# Autodesk Inventor assembly: Manfrotto Logo 01
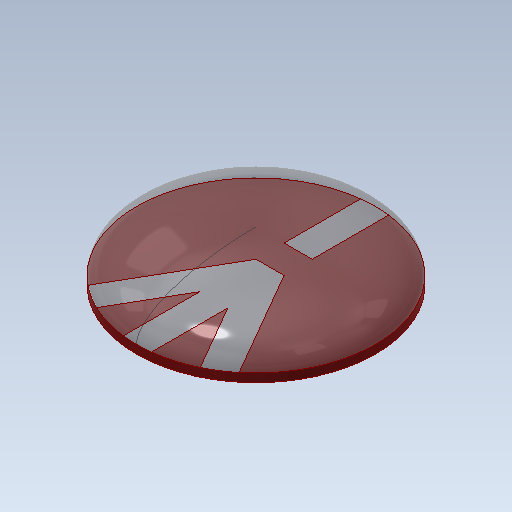
[picture p0: Inventor's stored thumbnail of the model, 512x512]
Saved by Autodesk Inventor 2020 (Build 240168000, 168)
## iProperties
Created: 2012-11-06
Part Number: Manfrotto Logo 01
Document SubType Name: Assembly
Designer: Lance
Mass: 0.140728 g
Surface Area: 2.47849 cm^2
Volume: 0.0737688 cm^3
Density: 1.90769 g/cm^3
Author: Lance
## Documents named in this file (3)
- C:\Users\Hesekiel\Desktop\MUM\Mechanika\Mechanizm elewacji i elektronika Filip\CAD\manfrotto-494rc2-tripod-head.snapshot.1\Manfrotto 494RC2 - Tripod Head\Manfrotto Logo 01.iam
- C:\Users\Hesekiel\Desktop\MUM\Mechanika\Mechanizm elewacji i elektronika Filip\CAD\manfrotto-494rc2-tripod-head.snapshot.1\Manfrotto 494RC2 - Tripod Head\Manfrotto Logo 01 - 1.ipt
- C:\Users\Hesekiel\Desktop\MUM\Mechanika\Mechanizm elewacji i elektronika Filip\CAD\manfrotto-494rc2-tripod-head.snapshot.1\Manfrotto 494RC2 - Tripod Head\Manfrotto Logo 01 - 2.ipt
## Components (2 placed, 2 different names)
1. Manfrotto Logo 01 - 1:1 — Insert:1, Angle:1
2. Manfrotto Logo 01 - 2:1 — Insert:1, Angle:1
## Relationships (2: Insert 1, Angle 1)
- Insert:1: Manfrotto Logo 01 - 1:1 ↔ Manfrotto Logo 01 - 2:1
- Angle:1 (180 deg): Manfrotto Logo 01 - 1:1 ↔ Manfrotto Logo 01 - 2:1
